# Autodesk Inventor assembly: VP-Dual-Redline
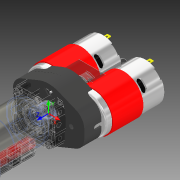
[picture p0: Inventor's stored thumbnail of the model, 180x180]
Saved by Autodesk Inventor 2021 (Build 250183000, 183)
## iProperties
Created: 2018-08-19
Part Number: VP-Dual-Redline
Document SubType Name: Assembly
Mass: 823.352 g
Surface Area: 940.04 cm^2
Volume: 140.134 cm^3
Density: 5.87546 g/cm^3
## Documents named in this file (15)
- D:\FIRST\Design\CollabPartsLib\Motors\FRC\Versaplanetary\V2 Stages\Dual Input Stage\VP Dual Redline Input.iam
- D:\FIRST\Design\CollabPartsLib\Motors\FRC\Versaplanetary\V2 Stages\Dual Input Housing.ipt
- D:\FIRST\Design\CollabPartsLib\Motors\FRC\Versaplanetary\V2 Stages\775pro Dual Input.ipt
- D:\FIRST\Design\CollabPartsLib\Motors\FRC\Versaplanetary\V2 Stages\Dual Input Alignment Pin.ipt
- D:\FIRST\Design\CollabPartsLib\Motors\FRC\Versaplanetary\Screws\8-32 Lock Nut.ipt
- D:\FIRST\Design\CollabPartsLib\Motors\FRC\Versaplanetary\Screws\8-32 x 0.75in Screw.ipt
- D:\FIRST\Design\CollabPartsLib\Motors\FRC\Versaplanetary\Screws\M4 x 10mm Screw.ipt
- D:\FIRST\Design\CollabPartsLib\Motors\FRC\Versaplanetary\V2 Stages\Dual Input Output Gear.ipt
- D:\FIRST\Design\CollabPartsLib\Motors\FRC\Versaplanetary\V2 Stages\Dual Input Coupler Gear.ipt
- D:\FIRST\Design\CollabPartsLib\Motors\FRC\Versaplanetary\Input Coupler\5mm Coupler Sleeve.ipt
- D:\FIRST\Design\CollabPartsLib\Motors\FRC\Versaplanetary\Input Coupler\Coupler Set Screw.ipt
- D:\FIRST\Design\CollabPartsLib\Motors\FRC\Redline.ipt
- D:\FIRST\Design\CollabPartsLib\Power Transfer\Bearings\6803ZZ.ipt
- D:\FIRST\Design\CollabPartsLib\Power Transfer\Bearings.ipt
- D:\FIRST\Design\CollabPartsLib\Motors\FRC\Versaplanetary\V2 Stages\Dual Input Stage.iam
## Components (22 placed, 12 different names)
1. Dual Input Housing:1 — Insert:3, Mate:1, Mate:2, Insert:4, Angle:1, Insert:5, Angle:2, Mate:3, Mate:8, Mate:15, Insert:38, Mate:16, Flush:3, Flush:4, Insert:39, Mate:17
2. 6803ZZ:1 — Insert:36, Insert:38
3. 775pro Dual Input:1 — Mate:1, Mate:2, Insert:6, Insert:11, Insert:12, Insert:13, Insert:14, Insert:20, Insert:21, Insert:22, Insert:23, Mate:15
4. 6803ZZ:2 — Insert:37
5. Dual Input Alignment Pin:1 — Insert:3
6. 8-32 Lock Nut:1 — Insert:4, Angle:1
7. 8-32 Lock Nut:2 — Insert:5, Angle:2
8. 8-32 x 0.75in Screw:1 — Insert:6, Flush:1, Mate:8
9. 8-32 x 0.75in Screw:2 — Mate:3, Flush:1
10. M4 x 10mm Screw:1 — Insert:11
11. M4 x 10mm Screw:2 — Insert:12
12. M4 x 10mm Screw:3 — Insert:13
13. M4 x 10mm Screw:4 — Insert:14
14. Dual Input Output Gear:1 — Rotation:1, Rotation:2, Insert:36, Insert:37
15. Dual Input Coupler Gear:1 — Insert:19, Rotation:2, Angle:4, Mate:5, Tangent:2, Mate:6, Flush:2
16. Dual Input Coupler Gear:2 — Insert:18, Rotation:1, Angle:3, Mate:4, Tangent:1, Mate:7, Flush:2, Insert:39
17. 5mm Coupler Sleeve:1 — Insert:18, Angle:3
18. 5mm Coupler Sleeve:2 — Insert:19, Angle:4, Insert:24, Mate:17
19. Coupler Set Screw:1 — Mate:4, Tangent:1
20. Coupler Set Screw:2 — Mate:5, Tangent:2
21. Redline:1 — Insert:20, Insert:22, Mate:6, Insert:24
22. Redline:2 — Insert:21, Insert:23, Mate:7
## Relationships (42: Insert 19, Mate 11, Angle 4, Flush 4, RelateRotation 2, Tangent 2)
- Insert:3: Dual Input Housing:1 ↔ Dual Input Alignment Pin:1
- Mate:1: Dual Input Housing:1 ↔ 775pro Dual Input:1
- Mate:2: Dual Input Housing:1 ↔ 775pro Dual Input:1
- Insert:4: Dual Input Housing:1 ↔ 8-32 Lock Nut:1
- Angle:1 (0 deg): Dual Input Housing:1 ↔ 8-32 Lock Nut:1
- Insert:5: Dual Input Housing:1 ↔ 8-32 Lock Nut:2
- Angle:2 (0 deg): Dual Input Housing:1 ↔ 8-32 Lock Nut:2
- Insert:6: 775pro Dual Input:1 ↔ 8-32 x 0.75in Screw:1
- Mate:3: Dual Input Housing:1 ↔ 8-32 x 0.75in Screw:2
- Flush:1: 8-32 x 0.75in Screw:1 ↔ 8-32 x 0.75in Screw:2
- Insert:11: 775pro Dual Input:1 ↔ M4 x 10mm Screw:1
- Insert:12: 775pro Dual Input:1 ↔ M4 x 10mm Screw:2
- Insert:13: 775pro Dual Input:1 ↔ M4 x 10mm Screw:3
- Insert:14: 775pro Dual Input:1 ↔ M4 x 10mm Screw:4
- Insert:18: Dual Input Coupler Gear:2 ↔ 5mm Coupler Sleeve:1
- Insert:19: Dual Input Coupler Gear:1 ↔ 5mm Coupler Sleeve:2
- Rotation:1 [RelateRotation] (1 ul): Dual Input Output Gear:1 ↔ Dual Input Coupler Gear:2
- Rotation:2 [RelateRotation] (1 ul): Dual Input Output Gear:1 ↔ Dual Input Coupler Gear:1
- Angle:3 (0 deg): Dual Input Coupler Gear:2 ↔ 5mm Coupler Sleeve:1
- Angle:4 (0 deg): Dual Input Coupler Gear:1 ↔ 5mm Coupler Sleeve:2
- Mate:4: Dual Input Coupler Gear:2 ↔ Coupler Set Screw:1
- Tangent:1: Dual Input Coupler Gear:2 ↔ Coupler Set Screw:1
- Mate:5: Dual Input Coupler Gear:1 ↔ Coupler Set Screw:2
- Tangent:2: Dual Input Coupler Gear:1 ↔ Coupler Set Screw:2
- Insert:20: 775pro Dual Input:1 ↔ Redline:1
- Insert:21: 775pro Dual Input:1 ↔ Redline:2
- Insert:22: 775pro Dual Input:1 ↔ Redline:1
- Insert:23: 775pro Dual Input:1 ↔ Redline:2
- Mate:6: Dual Input Coupler Gear:1 ↔ Redline:1
- Mate:7: Dual Input Coupler Gear:2 ↔ Redline:2
- Insert:24: 5mm Coupler Sleeve:2 ↔ Redline:1
- Mate:8: Dual Input Housing:1 ↔ 8-32 x 0.75in Screw:1
- Flush:2: Dual Input Coupler Gear:1 ↔ Dual Input Coupler Gear:2
- Mate:15: Dual Input Housing:1 ↔ 775pro Dual Input:1
- Insert:36: 6803ZZ:1 ↔ Dual Input Output Gear:1
- Insert:37: 6803ZZ:2 ↔ Dual Input Output Gear:1
- Insert:38: Dual Input Housing:1 ↔ 6803ZZ:1
- Mate:16: Dual Input Housing:1
- Flush:3: Dual Input Housing:1
- Flush:4: Dual Input Housing:1
- Insert:39: Dual Input Housing:1 ↔ Dual Input Coupler Gear:2
- Mate:17: Dual Input Housing:1 ↔ 5mm Coupler Sleeve:2
